# Autodesk Inventor assembly: SixWheelRobot
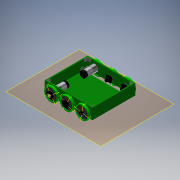
[picture p0: Inventor's stored thumbnail of the model, 180x180]
Saved by Autodesk Inventor 2018 (Build 220112000, 112)
## iProperties
Created: 2017-12-20
Part Number: SixWheelRobot
Document SubType Name: Assembly
Designer: jklei
Author: jklei
## Documents named in this file (13)
- C:\Users\jklei\Desktop\Projects\Shamrock\Hardware\SixWheelRobot.iam
- C:\Users\jklei\Desktop\Projects\Shamrock\Hardware\DriveRail.ipt
- C:\Users\jklei\Desktop\Projects\Shamrock\Hardware\SideRail.ipt
- C:\Users\jklei\Desktop\Projects\Shamrock\Hardware\251RPM-Motor.ipt
- C:\Users\jklei\Desktop\Projects\Shamrock\Hardware\BaneBots-T40-6mm-Shaft-Adapter.ipt
- C:\Users\jklei\Desktop\Projects\Shamrock\Hardware\BaneBots_Wheel.ipt
- C:\Users\jklei\Desktop\Projects\Shamrock\Hardware\Flanged_Bearing.ipt
- C:\Users\jklei\Desktop\Projects\Shamrock\Hardware\ScrewPlaceholder.ipt
- C:\Users\jklei\Desktop\Projects\Shamrock\Hardware\MellewellCornerBrace.ipt
- C:\Users\jklei\Desktop\Projects\Shamrock\Hardware\25_16-Tooth_Sprocket.ipt
- C:\Users\jklei\Desktop\Projects\Shamrock\Hardware\ThunderHex.ipt
- C:\Users\jklei\Desktop\Projects\Shamrock\Hardware\MotorShaft_ThunderHex.ipt
- C:\Users\jklei\Desktop\Projects\Shamrock\Hardware\ModBoard-Bottom.ipt
## Components (49 placed, 12 different names)
1. DriveRail:1 — Flush:1, Flush:2, Flush:5, Flush:6, Mate:2, Mate:3, Insert:2, Insert:7, Insert:8, Insert:9, Mate:5, Angle:2, Insert:12, Insert:15, Insert:17, Insert:18, Insert:24, Insert:27, Mate:41, Mate:42, Flush:11
2. DriveRail:2 — Flush:1, Flush:3, Flush:4, Flush:7, Mate:1, Insert:3, Insert:5, Insert:6, Insert:10, Mate:4, Insert:11, Insert:16, Angle:3, Insert:21, Angle:4, Insert:29, Mate:43, Mate:44
3. SideRail:1 — Flush:3, Flush:4, Flush:5, Mate:3, Mate:6, Insert:19, Insert:20, Insert:28, Flush:10, Mate:51, Mate:60, Flush:12, Insert:34, Insert:35
4. SideRail:2 — Flush:2, Flush:6, Flush:7, Mate:1, Mate:2, Angle:1, Insert:22, Insert:23, Insert:25, Insert:26, Insert:36, Insert:37
5. 251RPM-Motor:1 — Mate:5, Angle:2, Insert:12, Insert:13
6. 251RPM-Motor:2 — Angle:1, Mate:4, Insert:11, Insert:14
7. BaneBots-T40-6mm-Shaft-Adapter:1 — Insert:13, Mate:16, Mate:17, Mate:18, Angle:5, Mate:54
8. BaneBots-T40-6mm-Shaft-Adapter:2 — Insert:14, Mate:7, Mate:8, Mate:12, Angle:6, Mate:55
9. BaneBots_Wheel:1 — Mate:42, Angle:8, Mate:57
10. BaneBots_Wheel:2 — Mate:41, Mate:50, Angle:9, Mate:58
11. BaneBots_Wheel:3 — Mate:12, Mate:13, Angle:6, Mate:55
12. BaneBots_Wheel:4 — Mate:16, Mate:19, Angle:5, Mate:54
13. BaneBots_Wheel:5 — Mate:44, Angle:7, Mate:56
14. BaneBots_Wheel:6 — Mate:43, Mate:47, Angle:10, Mate:59
15. Flanged_Bearing:1 — Insert:3, Insert:31, Mate:46
16. Flanged_Bearing:2 — Insert:16, Insert:30, Mate:45
17. Flanged_Bearing:3 — Insert:15, Insert:32, Mate:49
18. Flanged_Bearing:4 — Insert:2, Insert:33, Mate:48
19. ScrewPlaceholder:1 — Insert:5
20. ScrewPlaceholder:2 — Insert:6
21. ScrewPlaceholder:3 — Insert:10
22. ScrewPlaceholder:4 — Insert:7
23. ScrewPlaceholder:5 — Insert:9
24. ScrewPlaceholder:6 — Insert:8
25. MellewellCornerBrace:1 — Insert:20, Angle:3
26. MellewellCornerBrace:2 — Insert:28, Insert:29
27. MellewellCornerBrace:3 — Insert:18, Insert:19
28. MellewellCornerBrace:4 — Insert:17, Mate:6
29. MellewellCornerBrace:5 — Insert:24, Insert:25
30. MellewellCornerBrace:6 — Insert:26, Insert:27
31. MellewellCornerBrace:7 — Insert:21, Insert:22
32. MellewellCornerBrace:8 — Insert:23, Angle:4
33. 25_16-Tooth_Sprocket:1 — Mate:7, Mate:8, Mate:13
34. 25_16-Tooth_Sprocket:2 — Mate:17, Mate:18, Mate:19
35. 25_16-Tooth_Sprocket:3 — Mate:31, Mate:32, Mate:48
36. 25_16-Tooth_Sprocket:4 — Mate:27, Mate:28, Mate:49
37. 25_16-Tooth_Sprocket:5 — Mate:25, Mate:29, Mate:50
38. 25_16-Tooth_Sprocket:6 — Mate:24, Mate:30, Mate:46
39. 25_16-Tooth_Sprocket:7 — Mate:22, Mate:23, Mate:45
40. 25_16-Tooth_Sprocket:8 — Mate:20, Mate:21, Mate:47
41. ThunderHex:1 — Insert:31, Mate:20, Mate:21, Mate:24, Mate:30, Angle:10, Mate:59
42. ThunderHex:2 — Insert:33, Mate:25, Mate:29, Mate:31, Mate:32, Angle:9, Mate:58
43. MotorShaft_ThunderHex:1 — Insert:32, Mate:27, Mate:28, Angle:8, Mate:57
44. MotorShaft_ThunderHex:2 — Insert:30, Mate:22, Mate:23, Angle:7, Mate:56
45. ModBoard-Bottom:1 — Flush:11, Mate:60, Flush:12, Angle:11, Angle:12, Angle:14, Angle:15, Mate:61, Angle:16
46. MellewellCornerBrace:9 — Insert:34, Angle:11
47. MellewellCornerBrace:10 — Insert:35, Angle:12
48. MellewellCornerBrace:11 — Insert:37, Angle:14, Angle:15, Mate:61
49. MellewellCornerBrace:12 — Insert:36, Angle:16
## Relationships (107: Mate 45, Insert 35, Angle 15, Flush 12)
- Flush:1: DriveRail:1 ↔ DriveRail:2
- Flush:2: DriveRail:1 ↔ SideRail:2
- Flush:3: DriveRail:2 ↔ SideRail:1
- Flush:4: DriveRail:2 ↔ SideRail:1
- Flush:5: DriveRail:1 ↔ SideRail:1
- Flush:6: DriveRail:1 ↔ SideRail:2
- Flush:7: DriveRail:2 ↔ SideRail:2
- Mate:1: DriveRail:2 ↔ SideRail:2
- Mate:2: DriveRail:1 ↔ SideRail:2
- Mate:3: DriveRail:1 ↔ SideRail:1
- Insert:2: DriveRail:1 ↔ Flanged_Bearing:4
- Insert:3: DriveRail:2 ↔ Flanged_Bearing:1
- Insert:5: DriveRail:2 ↔ ScrewPlaceholder:1
- Insert:6: DriveRail:2 ↔ ScrewPlaceholder:2
- Insert:7: DriveRail:1 ↔ ScrewPlaceholder:4
- Insert:8: DriveRail:1 ↔ ScrewPlaceholder:6
- Insert:9: DriveRail:1 ↔ ScrewPlaceholder:5
- Insert:10: DriveRail:2 ↔ ScrewPlaceholder:3
- Angle:1 (0 deg): SideRail:2 ↔ 251RPM-Motor:2
- Mate:4 (-44.45 mm): DriveRail:2 ↔ 251RPM-Motor:2
- Insert:11: DriveRail:2 ↔ 251RPM-Motor:2
- Mate:5 (-209.55 mm): DriveRail:1 ↔ 251RPM-Motor:1
- Angle:2 (0 deg): DriveRail:1 ↔ 251RPM-Motor:1
- Insert:12: DriveRail:1 ↔ 251RPM-Motor:1
- Insert:13 (1.5875 mm): 251RPM-Motor:1 ↔ BaneBots-T40-6mm-Shaft-Adapter:1
- Insert:14 (1.5875 mm): 251RPM-Motor:2 ↔ BaneBots-T40-6mm-Shaft-Adapter:2
- Insert:15: DriveRail:1 ↔ Flanged_Bearing:3
- Insert:16: DriveRail:2 ↔ Flanged_Bearing:2
- Insert:17: DriveRail:1 ↔ MellewellCornerBrace:4
- Mate:6: SideRail:1 ↔ MellewellCornerBrace:4
- Insert:18: DriveRail:1 ↔ MellewellCornerBrace:3
- Insert:19: SideRail:1 ↔ MellewellCornerBrace:3
- Insert:20: SideRail:1 ↔ MellewellCornerBrace:1
- Angle:3 (0 deg): DriveRail:2 ↔ MellewellCornerBrace:1
- Insert:21: DriveRail:2 ↔ MellewellCornerBrace:7
- Insert:22: SideRail:2 ↔ MellewellCornerBrace:7
- Insert:23: SideRail:2 ↔ MellewellCornerBrace:8
- Angle:4 (0 deg): DriveRail:2 ↔ MellewellCornerBrace:8
- Insert:24: DriveRail:1 ↔ MellewellCornerBrace:5
- Insert:25: SideRail:2 ↔ MellewellCornerBrace:5
- Insert:26: SideRail:2 ↔ MellewellCornerBrace:6
- Insert:27: DriveRail:1 ↔ MellewellCornerBrace:6
- Insert:28: SideRail:1 ↔ MellewellCornerBrace:2
- Insert:29: DriveRail:2 ↔ MellewellCornerBrace:2
- Mate:7: BaneBots-T40-6mm-Shaft-Adapter:2 ↔ 25_16-Tooth_Sprocket:1
- Mate:8: BaneBots-T40-6mm-Shaft-Adapter:2 ↔ 25_16-Tooth_Sprocket:1
- Mate:12: BaneBots-T40-6mm-Shaft-Adapter:2 ↔ BaneBots_Wheel:3
- Mate:13: BaneBots_Wheel:3 ↔ 25_16-Tooth_Sprocket:1
- Mate:16: BaneBots-T40-6mm-Shaft-Adapter:1 ↔ BaneBots_Wheel:4
- Mate:17: BaneBots-T40-6mm-Shaft-Adapter:1 ↔ 25_16-Tooth_Sprocket:2
- Mate:18: BaneBots-T40-6mm-Shaft-Adapter:1 ↔ 25_16-Tooth_Sprocket:2
- Mate:19: BaneBots_Wheel:4 ↔ 25_16-Tooth_Sprocket:2
- Flush:8
- Insert:30 (-19.05 mm): Flanged_Bearing:2 ↔ MotorShaft_ThunderHex:2
- Insert:31 (-25.4 mm): Flanged_Bearing:1 ↔ ThunderHex:1
- Insert:32 (-25.4 mm): Flanged_Bearing:3 ↔ MotorShaft_ThunderHex:1
- Insert:33 (-25.4 mm): Flanged_Bearing:4 ↔ ThunderHex:2
- Mate:20: 25_16-Tooth_Sprocket:8 ↔ ThunderHex:1
- Mate:21: 25_16-Tooth_Sprocket:8 ↔ ThunderHex:1
- Mate:22: 25_16-Tooth_Sprocket:7 ↔ MotorShaft_ThunderHex:2
- Mate:23: 25_16-Tooth_Sprocket:7 ↔ MotorShaft_ThunderHex:2
- Mate:24: 25_16-Tooth_Sprocket:6 ↔ ThunderHex:1
- Mate:25: 25_16-Tooth_Sprocket:5 ↔ ThunderHex:2
- Mate:27: 25_16-Tooth_Sprocket:4 ↔ MotorShaft_ThunderHex:1
- Mate:28: 25_16-Tooth_Sprocket:4 ↔ MotorShaft_ThunderHex:1
- Mate:29: 25_16-Tooth_Sprocket:5 ↔ ThunderHex:2
- Mate:30: 25_16-Tooth_Sprocket:6 ↔ ThunderHex:1
- Mate:31: 25_16-Tooth_Sprocket:3 ↔ ThunderHex:2
- Mate:32: 25_16-Tooth_Sprocket:3 ↔ ThunderHex:2
- Mate:41 (2.8575 mm): DriveRail:1 ↔ BaneBots_Wheel:2
- Mate:42 (2.8575 mm): DriveRail:1 ↔ BaneBots_Wheel:1
- Mate:43 (2.8575 mm): DriveRail:2 ↔ BaneBots_Wheel:6
- Mate:44 (2.8575 mm): DriveRail:2 ↔ BaneBots_Wheel:5
- Mate:45: Flanged_Bearing:2 ↔ 25_16-Tooth_Sprocket:7
- Mate:46: Flanged_Bearing:1 ↔ 25_16-Tooth_Sprocket:6
- Mate:47: BaneBots_Wheel:6 ↔ 25_16-Tooth_Sprocket:8
- Mate:48: Flanged_Bearing:4 ↔ 25_16-Tooth_Sprocket:3
- Mate:49: Flanged_Bearing:3 ↔ 25_16-Tooth_Sprocket:4
- Mate:50: BaneBots_Wheel:2 ↔ 25_16-Tooth_Sprocket:5
- Flush:9 (254 mm)
- Flush:10: SideRail:1
- Mate:51 (17.4752 mm): SideRail:1
- Angle:5 (0 deg): BaneBots-T40-6mm-Shaft-Adapter:1 ↔ BaneBots_Wheel:4
- Mate:54: BaneBots-T40-6mm-Shaft-Adapter:1 ↔ BaneBots_Wheel:4
- Angle:6 (0 deg): BaneBots-T40-6mm-Shaft-Adapter:2 ↔ BaneBots_Wheel:3
- Mate:55: BaneBots-T40-6mm-Shaft-Adapter:2 ↔ BaneBots_Wheel:3
- Angle:7 (0 deg): BaneBots_Wheel:5 ↔ MotorShaft_ThunderHex:2
- Mate:56: BaneBots_Wheel:5 ↔ MotorShaft_ThunderHex:2
- Angle:8 (0 deg): BaneBots_Wheel:1 ↔ MotorShaft_ThunderHex:1
- Mate:57: BaneBots_Wheel:1 ↔ MotorShaft_ThunderHex:1
- Angle:9 (0 deg): BaneBots_Wheel:2 ↔ ThunderHex:2
- Mate:58: BaneBots_Wheel:2 ↔ ThunderHex:2
- Angle:10 (0 deg): BaneBots_Wheel:6 ↔ ThunderHex:1
- Mate:59: BaneBots_Wheel:6 ↔ ThunderHex:1
- Flush:11 (28.575 mm): DriveRail:1 ↔ ModBoard-Bottom:1
- Mate:60: SideRail:1 ↔ ModBoard-Bottom:1
- Flush:12: SideRail:1 ↔ ModBoard-Bottom:1
- Insert:34: SideRail:1 ↔ MellewellCornerBrace:9
- Angle:11 (90 deg): ModBoard-Bottom:1 ↔ MellewellCornerBrace:9
- Insert:35: SideRail:1 ↔ MellewellCornerBrace:10
- Angle:12 (90 deg): ModBoard-Bottom:1 ↔ MellewellCornerBrace:10
- Insert:36: SideRail:2 ↔ MellewellCornerBrace:12
- Insert:37: SideRail:2 ↔ MellewellCornerBrace:11
- Angle:14 (90 deg): ModBoard-Bottom:1 ↔ MellewellCornerBrace:11
- Angle:15 (90 deg): ModBoard-Bottom:1 ↔ MellewellCornerBrace:11
- Mate:61: ModBoard-Bottom:1 ↔ MellewellCornerBrace:11
- Angle:16 (90 deg): ModBoard-Bottom:1 ↔ MellewellCornerBrace:12
